# Autodesk Inventor assembly: upper_w_head_fin1
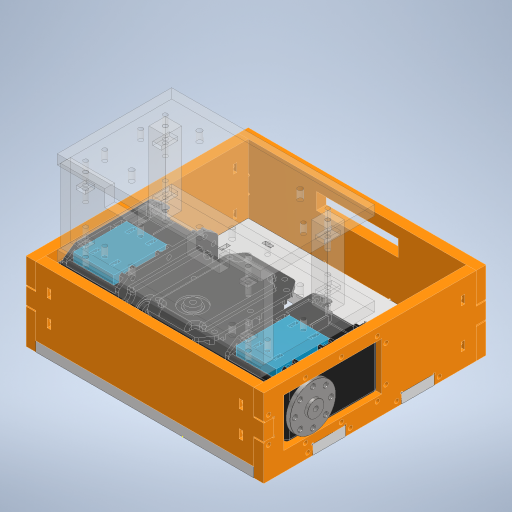
[picture p0: Inventor's stored thumbnail of the model, 512x512]
Saved by Autodesk Inventor 2024 (Build 280153000, 153)
## iProperties
Created: 2024-09-17
Part Number: upper_w_head_fin1
Document SubType Name: Assembly
Designer: jmha0
Author: jmha0
## Documents named in this file (3)
- C:\Users\jmha0\OneDrive\바탕 화면\19th_intern_hjm_fight_robot\부품\Upper_Body\Upper_w_head\upper_w_head_fin1.iam
- C:\Users\jmha0\OneDrive\바탕 화면\19th_intern_hjm_fight_robot\부품\Upper_Body\Upper\upper_fin1.iam
- C:\Users\jmha0\OneDrive\바탕 화면\19th_intern_hjm_fight_robot\부품\Upper_Body\head\head_fin1.iam
## Components (2 placed, 2 different names)
1. upper_fin1:1 [sub-assembly] — 삽입:1, 삽입:2
2. head_fin1:1 [sub-assembly] — 삽입:1, 삽입:2
## Relationships (2: Insert 2)
- 삽입:1 [Insert]: upper_fin1:1 ↔ head_fin1:1
- 삽입:2 [Insert]: upper_fin1:1 ↔ head_fin1:1
